# Autodesk Inventor assembly: MidShufflers
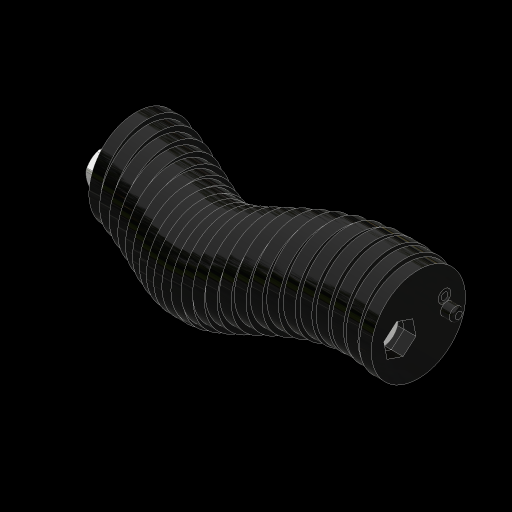
[picture p0: Inventor's stored thumbnail of the model, 512x512]
Saved by Autodesk Inventor 2023 (Build 270158000, 158)
## iProperties
Created: 2022-03-05
Part Number: MidShufflers
Document SubType Name: Assembly
Designer: tandu
Mass: 411.819 g
Surface Area: 1522.08 cm^2
Volume: 285.301 cm^3
Density: 1.44345 g/cm^3
Author: tandu
## Documents named in this file (7)
- C:\Users\tandu\Documents\GrabCAD\A Little Trolling\3 pound\MidShufflers.iam
- C:\Users\tandu\Documents\GrabCAD\A Little Trolling\3 pound\ShufflerBaseCam.ipt
- C:\Users\tandu\Documents\GrabCAD\A Little Trolling\3 pound\ShufflerMidCam.ipt
- C:\Users\tandu\Documents\GrabCAD\A Little Trolling\3 pound\ShufflerMidCam2.ipt
- C:\Users\tandu\Documents\GrabCAD\A Little Trolling\3 pound\ShufflerMidCam3.ipt
- C:\Users\tandu\Documents\GrabCAD\A Little Trolling\3 pound\ShufflerMidCam4.ipt
- C:\Users\tandu\Documents\GrabCAD\A Little Trolling\3 pound\3 inch 91115A852_Female Threaded Hex Standoff.ipt
## Components (26 placed, 6 different names)
1. ShufflerMidCam:6 — Insert:95, Flush:74, Insert:97, Flush:75
2. 3 inch 91115A852_Female Threaded Hex Standoff:1 — Mate:7, Mate:8, Mate:9
3. ShufflerBaseCam:1 — Mate:3, Insert:96, Mate:8
4. ShufflerMidCam3:6 — Insert:97, Flush:75
5. ShufflerMidCam2:1 — Insert:69, Flush:50, Insert:96
6. ShufflerMidCam4:1 — Insert:69, Flush:50, Insert:70, Flush:51
7. ShufflerMidCam:1 — Insert:70, Flush:51, Insert:71, Flush:52
8. ShufflerMidCam3:1 — Insert:71, Flush:52, Insert:72, Flush:53
9. ShufflerMidCam2:2 — Insert:72, Flush:53, Insert:73, Flush:54
10. ShufflerMidCam4:2 — Insert:73, Flush:54, Insert:74, Flush:55
11. ShufflerMidCam:2 — Insert:74, Flush:55, Insert:75, Flush:56
12. ShufflerMidCam3:2 — Insert:75, Flush:56, Insert:83, Flush:57
13. ShufflerMidCam2:3 — Insert:83, Flush:57, Flush:58
14. ShufflerMidCam4:3 — Flush:58, Flush:59
15. ShufflerMidCam:3 — Flush:59, Flush:60
16. ShufflerMidCam3:3 — Flush:60, Flush:61, Flush:62
17. ShufflerMidCam2:4 — Flush:61
18. ShufflerMidCam4:4 — Flush:62, Flush:63
19. ShufflerMidCam:4 — Flush:63, Flush:64
20. ShufflerMidCam3:4 — Flush:64, Insert:91, Flush:65
21. ShufflerMidCam2:5 — Insert:91, Flush:65, Flush:66
22. ShufflerMidCam4:5 — Flush:66, Flush:67
23. ShufflerMidCam:5 — Flush:67, Flush:68
24. ShufflerMidCam3:5 — Flush:68, Flush:69
25. ShufflerMidCam2:6 — Flush:69, Flush:70
26. ShufflerMidCam4:6 — Flush:70, Insert:95, Flush:74
## Relationships (53: Insert 24, Flush 23, Mate 6)
- Insert:69: ShufflerMidCam2:1 ↔ ShufflerMidCam4:1
- Flush:50: ShufflerMidCam2:1 ↔ ShufflerMidCam4:1
- Insert:70: ShufflerMidCam4:1 ↔ ShufflerMidCam:1
- Flush:51: ShufflerMidCam4:1 ↔ ShufflerMidCam:1
- Insert:71: ShufflerMidCam:1 ↔ ShufflerMidCam3:1
- Flush:52: ShufflerMidCam:1 ↔ ShufflerMidCam3:1
- Insert:72: ShufflerMidCam3:1 ↔ ShufflerMidCam2:2
- Flush:53: ShufflerMidCam3:1 ↔ ShufflerMidCam2:2
- Insert:73: ShufflerMidCam2:2 ↔ ShufflerMidCam4:2
- Flush:54: ShufflerMidCam2:2 ↔ ShufflerMidCam4:2
- Insert:74: ShufflerMidCam4:2 ↔ ShufflerMidCam:2
- Flush:55: ShufflerMidCam4:2 ↔ ShufflerMidCam:2
- Insert:75: ShufflerMidCam:2 ↔ ShufflerMidCam3:2
- Flush:56: ShufflerMidCam:2 ↔ ShufflerMidCam3:2
- [Insert]: ShufflerMidCam2:3 ↔ ShufflerMidCam4:3
- [Insert]: ShufflerMidCam4:3 ↔ ShufflerMidCam:3
- [Insert]: ShufflerMidCam:3 ↔ ShufflerMidCam3:3
- [Insert]: ShufflerMidCam3:3 ↔ ShufflerMidCam2:4
- [Insert]: ShufflerMidCam2:4 ↔ ShufflerMidCam4:4
- [Insert]: ShufflerMidCam4:4 ↔ ShufflerMidCam:4
- [Insert]: ShufflerMidCam:4 ↔ ShufflerMidCam3:4
- Insert:83: ShufflerMidCam3:2 ↔ ShufflerMidCam2:3
- Flush:57: ShufflerMidCam3:2 ↔ ShufflerMidCam2:3
- Flush:58: ShufflerMidCam2:3 ↔ ShufflerMidCam4:3
- Flush:59: ShufflerMidCam4:3 ↔ ShufflerMidCam:3
- Flush:60: ShufflerMidCam:3 ↔ ShufflerMidCam3:3
- Flush:61: ShufflerMidCam3:3 ↔ ShufflerMidCam2:4
- Flush:62: ShufflerMidCam3:3 ↔ ShufflerMidCam4:4
- Flush:63: ShufflerMidCam4:4 ↔ ShufflerMidCam:4
- Flush:64: ShufflerMidCam:4 ↔ ShufflerMidCam3:4
- [Insert]: ShufflerMidCam2:5 ↔ ShufflerMidCam4:5
- [Insert]: ShufflerMidCam4:5 ↔ ShufflerMidCam:5
- [Insert]: ShufflerMidCam:5 ↔ ShufflerMidCam3:5
- [Insert]: ShufflerMidCam3:5 ↔ ShufflerMidCam2:6
- [Insert]: ShufflerMidCam2:6 ↔ ShufflerMidCam4:6
- Insert:91: ShufflerMidCam3:4 ↔ ShufflerMidCam2:5
- Flush:65: ShufflerMidCam3:4 ↔ ShufflerMidCam2:5
- Flush:66: ShufflerMidCam2:5 ↔ ShufflerMidCam4:5
- Flush:67: ShufflerMidCam4:5 ↔ ShufflerMidCam:5
- Flush:68: ShufflerMidCam:5 ↔ ShufflerMidCam3:5
- Flush:69: ShufflerMidCam3:5 ↔ ShufflerMidCam2:6
- Flush:70: ShufflerMidCam2:6 ↔ ShufflerMidCam4:6
- Insert:95: ShufflerMidCam:6 ↔ ShufflerMidCam4:6
- Flush:74: ShufflerMidCam:6 ↔ ShufflerMidCam4:6
- Mate:3: ShufflerBaseCam:1
- [Mate]: 3 inch 91115A852_Female Threaded Hex Standoff:1 ↔ ShufflerBaseCam:1
- Insert:96: ShufflerBaseCam:1 ↔ ShufflerMidCam2:1
- [Mate]: 3 inch 91115A852_Female Threaded Hex Standoff:1 ↔ ShufflerMidCam2:1
- Mate:7: 3 inch 91115A852_Female Threaded Hex Standoff:1
- Mate:8: 3 inch 91115A852_Female Threaded Hex Standoff:1 ↔ ShufflerBaseCam:1
- Mate:9: 3 inch 91115A852_Female Threaded Hex Standoff:1
- Insert:97: ShufflerMidCam:6 ↔ ShufflerMidCam3:6
- Flush:75: ShufflerMidCam:6 ↔ ShufflerMidCam3:6
## Named parameters: d268_d254 = 0 mm, d269_d256 = 0 mm, d270_d258 = 0 mm, d271_d260 = 0 mm, d272_d262 = 0 mm, d273_d264 = 0 mm, d274_d266 = 0 mm, d284_d268_d254 = 0 mm, d285_d269_d256 = 0 mm, d286_d270_d258 = 0 mm, d287_d271_d260 = 0 mm, d288_d272_d262 = 0 mm
